# Autodesk Inventor assembly: ToolHolderAdapterAssy
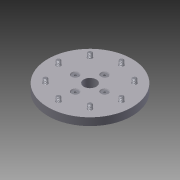
[picture p0: Inventor's stored thumbnail of the model, 180x180]
Saved by Autodesk Inventor 2012 SP1 (Build 160190100, 190)
## iProperties
Created: 2010-03-22
Part Number: ToolHolderAdapterAssy
Document SubType Name: Assembly
Designer: rconnaug
Author: rconnaug
## Documents named in this file (5)
- D:\Users\ding42\Dropbox\Inventor files\CMS\Module Assembly Station\Gantry\NewGantryParts\NewParts\ToolHolderAdapter\ToolHolderAdapterAssy.iam
- D:\Users\ding42\Dropbox\Inventor files\CMS\Module Assembly Station\Gantry\NewGantryParts\NewParts\ToolHolderAdapter\ToolHolderAdapter.ipt
- D:\Users\ding42\Dropbox\Inventor files\CMS\Module Assembly Station\Gantry\NewGantryParts\NewParts\ToolHolderAdapter\92125A211.ipt
- D:\Users\ding42\Dropbox\Inventor files\CMS\Module Assembly Station\Gantry\NewGantryParts\NewParts\ToolHolderAdapter\92210A151.ipt
- D:\Users\ding42\Dropbox\Inventor files\CMS\Module Assembly Station\Gantry\NewGantryParts\NewParts\ToolHolderAdapter\9262K645 Buna-N O-Ring .ipt
## Components (14 placed, 4 different names)
1. ToolHolderAdapter:1 — Mate:6, Mate:7, Mate:9, Mate:10, Mate:11, Mate:15, Mate:16, Mate:17, Mate:18, Mate:19, Mate:20, Mate:21, Insert:1
2. 92125A211:1 — Mate:6
3. 92210A151:1 — Mate:7
4. 92125A211:2 — Mate:20
5. 92125A211:3 — Mate:18
6. 92125A211:4 — Mate:19
7. 92125A211:5 — Mate:17
8. 92125A211:7 — Mate:16
9. 92125A211:8 — Mate:15
10. 92210A151:2 — Mate:10
11. 92210A151:3 — Mate:9
12. 92210A151:4 — Mate:11
13. 92125A211:9 — Mate:21
14. 9262K645 Buna-N O-Ring :1 — Insert:1
## Relationships (13: Mate 12, Insert 1)
- Mate:6: ToolHolderAdapter:1 ↔ 92125A211:1
- Mate:7: ToolHolderAdapter:1 ↔ 92210A151:1
- Mate:9: ToolHolderAdapter:1 ↔ 92210A151:3
- Mate:10: ToolHolderAdapter:1 ↔ 92210A151:2
- Mate:11: ToolHolderAdapter:1 ↔ 92210A151:4
- Mate:15: ToolHolderAdapter:1 ↔ 92125A211:8
- Mate:16: ToolHolderAdapter:1 ↔ 92125A211:7
- Mate:17: ToolHolderAdapter:1 ↔ 92125A211:5
- Mate:18: ToolHolderAdapter:1 ↔ 92125A211:3
- Mate:19: ToolHolderAdapter:1 ↔ 92125A211:4
- Mate:20: ToolHolderAdapter:1 ↔ 92125A211:2
- Mate:21: ToolHolderAdapter:1 ↔ 92125A211:9
- Insert:1: ToolHolderAdapter:1 ↔ 9262K645 Buna-N O-Ring :1
